# Autodesk Inventor assembly: Assembly Mec 2.0 side
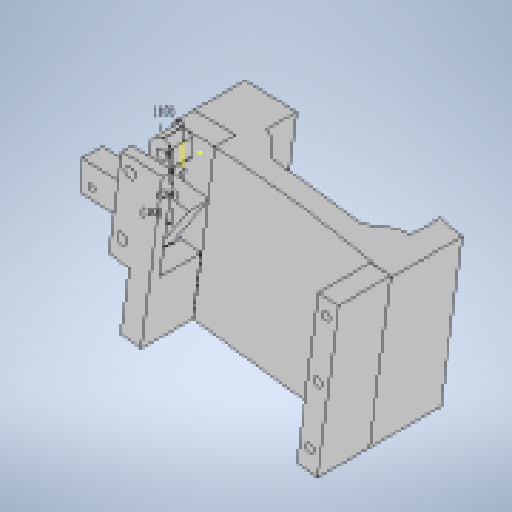
[picture p0: Inventor's stored thumbnail of the model, 512x512]
Saved by Autodesk Inventor 2025 (Build 290162000, 162)
## iProperties
Created: 2025-11-13
Part Number: Assembly Mec 2.0 side
Document SubType Name: Assembly
Designer: ruven
Author: ruven
## Documents named in this file (7)
- C:\Users\ruven\OneDrive\Dokumente\Uni\MCI\Semester 3\student project\Assembly Mec 2.0 side.iam
- C:\Users\ruven\OneDrive\Dokumente\Uni\MCI\Semester 3\student project\ReleaseMec2.0TopPlate.ipt
- C:\Users\ruven\OneDrive\Dokumente\Uni\MCI\Semester 3\student project\ReleaseMec2.0SideWall.ipt
- C:\Users\ruven\OneDrive\Dokumente\Uni\MCI\Semester 3\student project\ReleaseMec2.0SideMec.ipt
- C:\Users\ruven\OneDrive\Dokumente\Uni\MCI\Semester 3\student project\HoldingPin.ipt
- C:\Users\ruven\OneDrive\Dokumente\Uni\MCI\Semester 3\student project\ReleasePin.ipt
- C:\Users\ruven\OneDrive\Dokumente\Uni\MCI\Semester 3\student project\HoldingTri.ipt
## Components (6 placed, 6 different names)
1. ReleaseMec2.0TopPlate:1 — Mate:1, Mate:2, Mate:3, Mate:4, Mate:5, Mate:6
2. ReleaseMec2.0SideWall:1 — Mate:1, Mate:2, Mate:3
3. ReleaseMec2.0SideMec:1 — Mate:4, Mate:5, Mate:6, Mate:7, Mate:8, Mate:11, Mate:12, Mate:13, Mate:14
4. HoldingPin:1 — Mate:7, Mate:8
5. ReleasePin:1 — Mate:11, Mate:12
6. HoldingTri:1 — Mate:13, Mate:14
## Relationships (12: Mate 12)
- Mate:1: ReleaseMec2.0TopPlate:1 ↔ ReleaseMec2.0SideWall:1
- Mate:2: ReleaseMec2.0TopPlate:1 ↔ ReleaseMec2.0SideWall:1
- Mate:3: ReleaseMec2.0TopPlate:1 ↔ ReleaseMec2.0SideWall:1
- Mate:4: ReleaseMec2.0TopPlate:1 ↔ ReleaseMec2.0SideMec:1
- Mate:5: ReleaseMec2.0TopPlate:1 ↔ ReleaseMec2.0SideMec:1
- Mate:6: ReleaseMec2.0TopPlate:1 ↔ ReleaseMec2.0SideMec:1
- Mate:7: ReleaseMec2.0SideMec:1 ↔ HoldingPin:1
- Mate:8: ReleaseMec2.0SideMec:1 ↔ HoldingPin:1
- Mate:11: ReleaseMec2.0SideMec:1 ↔ ReleasePin:1
- Mate:12: ReleaseMec2.0SideMec:1 ↔ ReleasePin:1
- Mate:13: ReleaseMec2.0SideMec:1 ↔ HoldingTri:1
- Mate:14: ReleaseMec2.0SideMec:1 ↔ HoldingTri:1
